# Autodesk Inventor assembly: Assembly Light Stack
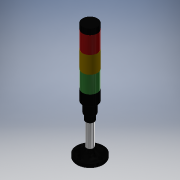
[picture p0: Inventor's stored thumbnail of the model, 180x180]
Saved by Autodesk Inventor 2017 (Build 210142000, 142)
## iProperties
Created: 2020-05-28
Part Number: Assembly Light Stack
Document SubType Name: Assembly
Designer: Sid
Author: Sid
## Documents named in this file (5)
- G:\My Drive\Rotary Inspection Machine v1\rotary-optical-sorting-cad\Electrical\Stack Light\Assembly Light Stack.iam
- G:\My Drive\Rotary Inspection Machine v1\rotary-optical-sorting-cad\Electrical\Stack Light\Light Stack.ipt
- G:\My Drive\Rotary Inspection Machine v1\rotary-optical-sorting-cad\Electrical\Stack Light\Connecting Rod.ipt
- G:\My Drive\Rotary Inspection Machine v1\rotary-optical-sorting-cad\Electrical\Stack Light\Base.ipt
- G:\My Drive\Rotary Inspection Machine v1\rotary-optical-sorting-cad\Electrical\Stack Light\Black Rubber Pad Bottom.ipt
## Components (4 placed, 4 different names)
1. Light Stack:1 — Cylindrical:1
2. Connecting Rod:1 — Cylindrical:1, Rotational:1
3. Base:1 — Rotational:1, Rotational:2
4. Black Rubber Pad Bottom:1 — Rotational:2
## Relationships (3: RevoluteJoint 2, CylindricalJoint 1)
- Cylindrical:1: Light Stack:1 ↔ Connecting Rod:1
- Rotational:1 [RevoluteJoint]: Connecting Rod:1 ↔ Base:1
- Rotational:2 [RevoluteJoint]: Base:1 ↔ Black Rubber Pad Bottom:1
